# Autodesk Inventor assembly: Assembly_SO-OCT_v0
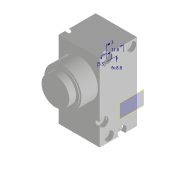
[picture p0: Inventor's stored thumbnail of the model, 180x180]
Saved by Autodesk Inventor 2022 (Build 260153000, 153)
## iProperties
Created: 2023-01-02
Part Number: Assembly_SO-OCT_v0
Document SubType Name: Assembly
Designer: diederichbenedict
Author: diederichbenedict
## Documents named in this file (13)
- C:\Users\diederichbenedict\Dropbox\Dokumente\Promotion\PROJECTS\SO-OCT\INVENTOR\Assembly_SO-OCT_v0.iam
- C:\Users\diederichbenedict\Dropbox\Dokumente\Promotion\PROJECTS\SO-OCT\INVENTOR\00_10x_Objective_ViewSolutions_bm05073332.ipt
- C:\Users\diederichbenedict\Dropbox\Dokumente\Promotion\PROJECTS\SO-OCT\INVENTOR\00_BS_KES400A_4mm.ipt
- C:\Users\diederichbenedict\Dropbox\Dokumente\Promotion\PROJECTS\SO-OCT\INVENTOR\00_VCM_M12.ipt
- C:\Users\diederichbenedict\Dropbox\Dokumente\Promotion\PROJECTS\SO-OCT\INVENTOR\00_Magnet_8x3mm.ipt
- C:\Users\diederichbenedict\Dropbox\Dokumente\Promotion\PROJECTS\SO-OCT\INVENTOR\00_F3SS25-Step.ipt
- C:\Users\diederichbenedict\Dropbox\Dokumente\Promotion\PROJECTS\SO-OCT\INVENTOR\00_F3SSN1P-Step.ipt
- C:\Users\diederichbenedict\Dropbox\Dokumente\Promotion\PROJECTS\SO-OCT\INVENTOR\01_optical_beam_path.ipt
- C:\Users\diederichbenedict\Dropbox\Dokumente\Promotion\PROJECTS\SO-OCT\INVENTOR\00_mirror_tmp.ipt
- C:\Users\diederichbenedict\Dropbox\Dokumente\Promotion\PROJECTS\SO-OCT\INVENTOR\10_SOOCT_Base_v0.ipt
- C:\Users\diederichbenedict\Dropbox\Dokumente\Promotion\PROJECTS\SO-OCT\INVENTOR\10_SOOCT_VCM_Mount_v0.ipt
- C:\Users\diederichbenedict\Dropbox\Dokumente\Promotion\PROJECTS\SO-OCT\INVENTOR\10_SOOCT_Base_v0_MIR.ipt
- C:\Users\diederichbenedict\Dropbox\Dokumente\Promotion\PROJECTS\SO-OCT\INVENTOR\tmp_20_Cube_Insert_Kinematic_Astromedia_30x40x90_pro_magnetic_M12lens_mirrormount.ipt
## Components (16 placed, 12 different names)
1. 00_10x_Objective_ViewSolutions_bm05073332:1 — Fluchtend:1, Fluchtend:2, Fluchtend:3, Fluchtend:4, Fluchtend:5, Passend:9
2. 00_VCM_M12:1 — Passend:5, Passend:6, Fluchtend:5, Fluchtend:6, Fluchtend:7, Einfügen:7
3. 01_optical_beam_path:1 — Fluchtend:1, Passend:1, Passend:2, Passend:3, Passend:5, Passend:9, Passend:10, Passend:11
4. 00_mirror_tmp:1 — Fluchtend:2, Fluchtend:3, Passend:1
5. 00_mirror_tmp:2 — Fluchtend:4, Passend:2, Passend:3, Passend:6
6. 00_BS_KES400A_4mm:1 — Passend:10, Passend:11
7. 10_SOOCT_Base_v0:1 — Fluchtend:6
8. 10_SOOCT_VCM_Mount_v0:1 — Fluchtend:7, Einfügen:6, Passend:12, Passend:14
9. 00_Magnet_8x3mm:3 — Einfügen:6
10. 00_F3SSN1P-Step:3 — Passend:13
11. 00_F3SS25-Step:3 — Passend:12, Passend:13
12. 00_F3SS25-Step:4 — Passend:14, Passend:15
13. 00_F3SSN1P-Step:4 — Passend:15
14. 10_SOOCT_Base_v0_MIR:1 — Einfügen:8
15. tmp_20_Cube_Insert_Kinematic_Astromedia_30x40x90_pro_magnetic_M12lens_mirrormount:1 — Einfügen:7
16. 00_Magnet_8x3mm:4 — Einfügen:8
## Relationships (22: Mate 12, Flush 7, Insert 3)
- Fluchtend:1 [Flush]: 00_10x_Objective_ViewSolutions_bm05073332:1 ↔ 01_optical_beam_path:1
- Fluchtend:2 [Flush]: 00_10x_Objective_ViewSolutions_bm05073332:1 ↔ 00_mirror_tmp:1
- Fluchtend:3 [Flush]: 00_10x_Objective_ViewSolutions_bm05073332:1 ↔ 00_mirror_tmp:1
- Passend:1 [Mate]: 01_optical_beam_path:1 ↔ 00_mirror_tmp:1
- Fluchtend:4 [Flush]: 00_10x_Objective_ViewSolutions_bm05073332:1 ↔ 00_mirror_tmp:2
- Passend:2 [Mate]: 01_optical_beam_path:1 ↔ 00_mirror_tmp:2
- Passend:3 [Mate]: 01_optical_beam_path:1 ↔ 00_mirror_tmp:2
- Passend:5 [Mate] (2 mm): 00_VCM_M12:1 ↔ 01_optical_beam_path:1
- Passend:6 [Mate] (6 mm): 00_VCM_M12:1 ↔ 00_mirror_tmp:2
- Fluchtend:5 [Flush]: 00_10x_Objective_ViewSolutions_bm05073332:1 ↔ 00_VCM_M12:1
- Passend:9 [Mate]: 00_10x_Objective_ViewSolutions_bm05073332:1 ↔ 01_optical_beam_path:1
- Passend:10 [Mate]: 01_optical_beam_path:1 ↔ 00_BS_KES400A_4mm:1
- Passend:11 [Mate]: 01_optical_beam_path:1 ↔ 00_BS_KES400A_4mm:1
- Fluchtend:6 [Flush] (8 mm): 00_VCM_M12:1 ↔ 10_SOOCT_Base_v0:1
- Fluchtend:7 [Flush]: 00_VCM_M12:1 ↔ 10_SOOCT_VCM_Mount_v0:1
- Einfügen:6 [Insert]: 10_SOOCT_VCM_Mount_v0:1 ↔ 00_Magnet_8x3mm:3
- Passend:12 [Mate]: 10_SOOCT_VCM_Mount_v0:1 ↔ 00_F3SS25-Step:3
- Passend:13 [Mate]: 00_F3SSN1P-Step:3 ↔ 00_F3SS25-Step:3
- Passend:14 [Mate]: 10_SOOCT_VCM_Mount_v0:1 ↔ 00_F3SS25-Step:4
- Passend:15 [Mate]: 00_F3SS25-Step:4 ↔ 00_F3SSN1P-Step:4
- Einfügen:7 [Insert] (0.1 mm): 00_VCM_M12:1 ↔ tmp_20_Cube_Insert_Kinematic_Astromedia_30x40x90_pro_magnetic_M12lens_mirrormount:1
- Einfügen:8 [Insert]: 10_SOOCT_Base_v0_MIR:1 ↔ 00_Magnet_8x3mm:4
